# Autodesk Inventor assembly: EnsambleTuberiaEntradaAire
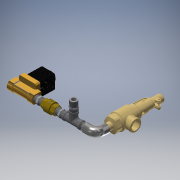
[picture p0: Inventor's stored thumbnail of the model, 180x180]
Saved by Autodesk Inventor 2017 (Build 210142000, 142)
## iProperties
Created: 2021-06-28
Part Number: EnsambleTuberiaEntradaAire
Document SubType Name: Assembly
Designer: USUARIO
Author: USUARIO
## Documents named in this file (7)
- D:\Laboratorio\Autoclave\Autoclave Horizontal\Con Precamara\2021\Autoclave 110L Biocacol OP2021110 #0045886XX\Modelo\EnsambleTuberiaEntradaAire.iam
- C:\Modelos 3D y DXF\Racores\B122 1-2x1-2.ipt
- C:\Modelos 3D y DXF\Racores\User Library-Tee_Class300.ipt
- C:\Modelos 3D y DXF\Racores\CodoCalle.iam
- C:\Modelos 3D y DXF\Racores\User Library-Valvula-segur-popup-1-2.ipt
- C:\Modelos 3D y DXF\Racores\Check Valve 0.5.ipt
- C:\Modelos 3D y DXF\Danfoss EV210B\DANFOS EV225B.ipt
## Components (8 placed, 6 different names)
1. B122 1-2x1-2:1
2. User Library-Tee_Class300:1
3. CodoCalle:1 [sub-assembly]
4. User Library-Valvula-segur-popup-1-2:1
5. B122 1-2x1-2:2
6. Check Valve 0.5:1
7. B122 1-2x1-2:3
8. DANFOS EV225B:1
## Relationships (7: Insert 7)
- [Insert] (9 mm): B122 1-2x1-2:1 ↔ User Library-Tee_Class300:1
- [Insert] (-10 mm): User Library-Tee_Class300:1 ↔ CodoCalle:1
- [Insert] (-9 mm): CodoCalle:1 ↔ User Library-Valvula-segur-popup-1-2:1
- [Insert] (-9 mm): User Library-Tee_Class300:1 ↔ B122 1-2x1-2:2
- [Insert] (-7 mm): B122 1-2x1-2:2 ↔ Check Valve 0.5:1
- [Insert] (-7 mm): Check Valve 0.5:1 ↔ B122 1-2x1-2:3
- [Insert] (-9 mm): B122 1-2x1-2:3 ↔ DANFOS EV225B:1
## Named parameters: d0_d6 = -9 mm
